# Autodesk Inventor assembly: Blower
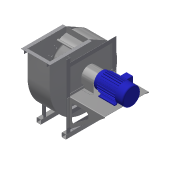
[picture p0: Inventor's stored thumbnail of the model, 180x180]
Saved by Autodesk Inventor 2022 (Build 260148000, 148)
## iProperties
Created: 2013-05-01
Part Number: Blower
Description: BOM Description
Document SubType Name: Assembly
Designer: user
Stock Number: N/A
HEAT TREAT: N/A
TOOL CODE: N/A
YEAR: 2012
Title: TITLE
Subject: SUB-TITLE
Author: user
## Documents named in this file (8)
- D:\Autodesk Inventor 2021 Advanced Assembly Modeling Practice Files\Blower\Blower.iam
- D:\Autodesk Inventor 2021 Advanced Assembly Modeling Practice Files\Blower\fan with wheel.iam
- D:\Autodesk Inventor 2021 Advanced Assembly Modeling Practice Files\Blower\TEFC NEMA, 286TS.ipt
- C:\Users\user\ProjectTemp\CML Northern Blower\TEFC NEMA Motor\TEFC NEMA Motor.ipt
- D:\Autodesk Inventor 2021 Advanced Assembly Modeling Practice Files\Blower\Coupler.ipt
- D:\Autodesk Inventor 2021 Advanced Assembly Modeling Practice Files\Blower\Guard, Shaft.ipt
- D:\Autodesk Inventor 2021 Advanced Assembly Modeling Practice Files\Blower\AISC - 3.5x3.5x3_16 - 40.ipt
- D:\Autodesk Inventor 2021 Advanced Assembly Modeling Practice Files\Blower\Mount_Blower.ipt
## Components (7 placed, 6 different names)
1. fan with wheel:1 [sub-assembly] — Insert:1, Angle:1, Flush:1, Mate:3, Mate:4, Mate:7, Mate:8, Flush:2, Flush:4
2. TEFC NEMA, 286TS:1 — Insert:2, Angle:1, Mate:2, Mate:6
3. Coupler:1 — Insert:1, Insert:2
4. Mount_Blower:1 — Flush:1, Mate:2, Mate:3, Mate:5, Flush:5
5. Guard, Shaft:1 — Mate:4, Mate:5, Mate:6
6. AISC - 3.5x3.5x3_16 - 40:1 — Mate:7, Flush:2, Flush:3
7. AISC - 3.5x3.5x3_16 - 40:2 — Mate:8, Flush:3, Flush:4, Flush:5
## Relationships (15: Mate 7, Flush 5, Insert 2, Angle 1)
- Insert:1: fan with wheel:1 ↔ Coupler:1
- Insert:2: TEFC NEMA, 286TS:1 ↔ Coupler:1
- Angle:1 (0 deg): fan with wheel:1 ↔ TEFC NEMA, 286TS:1
- Flush:1: fan with wheel:1 ↔ Mount_Blower:1
- Mate:2: TEFC NEMA, 286TS:1 ↔ Mount_Blower:1
- Mate:3: fan with wheel:1 ↔ Mount_Blower:1
- Mate:4: fan with wheel:1 ↔ Guard, Shaft:1
- Mate:5: Mount_Blower:1 ↔ Guard, Shaft:1
- Mate:6: TEFC NEMA, 286TS:1 ↔ Guard, Shaft:1
- Mate:7: fan with wheel:1 ↔ AISC - 3.5x3.5x3_16 - 40:1
- Mate:8: fan with wheel:1 ↔ AISC - 3.5x3.5x3_16 - 40:2
- Flush:2: fan with wheel:1 ↔ AISC - 3.5x3.5x3_16 - 40:1
- Flush:3: AISC - 3.5x3.5x3_16 - 40:1 ↔ AISC - 3.5x3.5x3_16 - 40:2
- Flush:4: fan with wheel:1 ↔ AISC - 3.5x3.5x3_16 - 40:2
- Flush:5 (15.875 mm): Mount_Blower:1 ↔ AISC - 3.5x3.5x3_16 - 40:2
